# Autodesk Inventor assembly: 1311-0016-1006 assembly
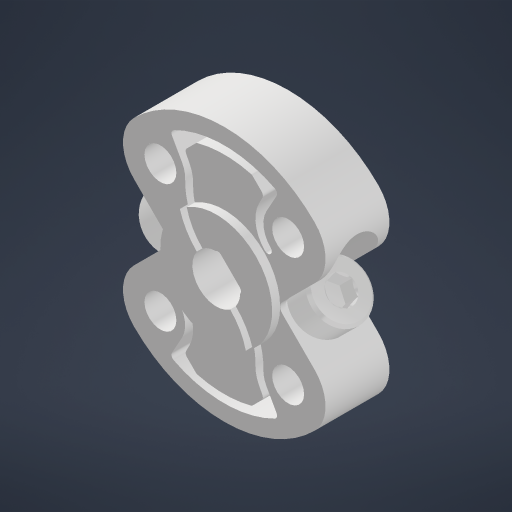
[picture p0: Inventor's stored thumbnail of the model, 512x512]
Saved by Autodesk Inventor 2023 (Build 270158000, 158)
## iProperties
Created: 2019-12-17
Part Number: 1311-0016-1006 assembly
Description: STEP AP203
Document SubType Name: Assembly
Designer: Arash
Sending System: SolidWorks 2016
Preprocessor: SwSTEP 2.0
Title: 1311-0016-1006 assembly.STEP
Revision Number: ANY
## Documents named in this file (3)
- C:\$WorkingFolder\Engineering Data\FTC_Parts_Library\goBilda\Motion\Hubs\Sonic Hubs\Thru-Hole Sonic Hub (6mm D-Bore).iam
- C:\$WorkingFolder\Engineering Data\FTC_Parts_Library\goBilda\Motion\Hubs\Sonic Hubs\1311-0016-1006.ipt
- C:\$WorkingFolder\Engineering Data\FTC_Parts_Library\ISO Standard Hardware\Screws\Sockethead Screws\Cap Screws\M4 x 0.7mm\(M4 x 0.7 x 14) Sockethead Cap Screw.ipt
## Components (3 placed, 2 different names)
1. 1311-0016-1006_1 — Mate:1, Mate:2, Mate:3, Mate:4
2. (M4 x 0.7 x 14) Sockethead Cap Screw:1 — Mate:1, Mate:2
3. (M4 x 0.7 x 14) Sockethead Cap Screw:2 — Mate:3, Mate:4
## Relationships (4: Mate 4)
- Mate:1: 1311-0016-1006_1 ↔ (M4 x 0.7 x 14) Sockethead Cap Screw:1
- Mate:2: 1311-0016-1006_1 ↔ (M4 x 0.7 x 14) Sockethead Cap Screw:1
- Mate:3: 1311-0016-1006_1 ↔ (M4 x 0.7 x 14) Sockethead Cap Screw:2
- Mate:4: 1311-0016-1006_1 ↔ (M4 x 0.7 x 14) Sockethead Cap Screw:2
